# Autodesk Inventor assembly: NUEVO Ensamble de estructura H
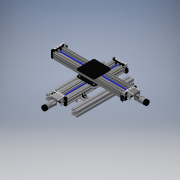
[picture p0: Inventor's stored thumbnail of the model, 180x180]
Saved by Autodesk Inventor 2018.3 (Build 223284000, 284)
## iProperties
Created: 2020-12-03
Part Number: NUEVO Ensamble de estructura H
Material: Genérico
Description: STEP AP203
Document SubType Name: Assembly
Designer: SERGIO ROMO
Sending System: SolidWorks 2019
Preprocessor: SwSTEP 2.0
Title: Ensamble del Arreglo.STEP
Revision Number: ANY
## Documents named in this file (23)
- C:\Users\SERGIO ROMO\Documents\GitHub\RemBot\CAD\Balanceo de masa\Inventor\NUEVO Ensamble de estructura H.iam
- C:\Users\SERGIO ROMO\Documents\GitHub\RemBot\CAD\Balanceo de masa\Inventor\C-Beam Actuator Lineal 500mm (Sin motor, sin carrito).ipt
- C:\Users\SERGIO ROMO\Documents\GitHub\RemBot\CAD\Balanceo de masa\Inventor\XLarge C-Beam Gantry Kit.iam
- C:\Users\SERGIO ROMO\Documents\GitHub\RemBot\CAD\Balanceo de masa\Inventor\Perfil de Aluminio.ipt
- C:\Users\SERGIO ROMO\Documents\GitHub\RemBot\CAD\Balanceo de masa\Inventor\Clavo.ipt
- C:\Users\SERGIO ROMO\Documents\GitHub\RemBot\CAD\Balanceo de masa\Inventor\Gearmotor_37D_19a1.ipt
- C:\Users\SERGIO ROMO\Documents\GitHub\RemBot\CAD\Balanceo de masa\Inventor\Impresion3D.ipt
- C:\Users\SERGIO ROMO\Documents\GitHub\RemBot\CAD\Balanceo de masa\Inventor\C-Beam Gantry Plate XLarge.step.ipt
- C:\Users\SERGIO ROMO\Documents\GitHub\RemBot\CAD\Balanceo de masa\Inventor\Bracket Inventor.ipt
- C:\Users\SERGIO ROMO\Documents\GitHub\RemBot\CAD\Balanceo de masa\Inventor\KW8-2.ipt
- C:\Users\SERGIO ROMO\Documents\GitHub\RemBot\CAD\Balanceo de masa\Inventor\Impresion3D sin Bracket.ipt
- C:\Users\SERGIO ROMO\Documents\GitHub\RemBot\CAD\Balanceo de masa\Inventor\Clavo de Arriba.ipt
- C:\Users\SERGIO ROMO\Documents\GitHub\RemBot\CAD\Balanceo de masa\Inventor\Tornillo final de carrera.ipt
- C:\Users\SERGIO ROMO\Documents\GitHub\RemBot\CAD\Balanceo de masa\Inventor\Perfil de Aluminio corta.ipt
- C:\Users\SERGIO ROMO\Documents\GitHub\RemBot\CAD\Balanceo de masa\Inventor\Triangulo.ipt
- C:\Users\SERGIO ROMO\Documents\GitHub\RemBot\CAD\Balanceo de masa\Inventor\TornilloM6.ipt
- C:\Users\SERGIO ROMO\Documents\GitHub\RemBot\CAD\Balanceo de masa\Inventor\Tuerca para tornilloM6.ipt
- C:\Users\SERGIO ROMO\Documents\GitHub\RemBot\CAD\Balanceo de masa\Inventor\Sujetador.ipt
- C:\Users\SERGIO ROMO\Documents\GitHub\RemBot\CAD\Balanceo de masa\Inventor\TornilloM8.ipt
- C:\Users\SERGIO ROMO\Documents\GitHub\RemBot\CAD\Balanceo de masa\Inventor\Tuerca para tornilloM8.ipt
- C:\Users\SERGIO ROMO\Documents\GitHub\RemBot\CAD\Balanceo de masa\Inventor\Tornillo para Bracket.ipt
- C:\Users\SERGIO ROMO\Documents\GitHub\RemBot\CAD\Balanceo de masa\Inventor\Tornillo para Motor Pololu.ipt
- C:\Users\SERGIO ROMO\Documents\GitHub\RemBot\CAD\Balanceo de masa\Inventor\Husillo 400 mm.ipt
## Components (100 placed, 27 different names)
1. XLarge C-Beam Gantry Kit_2 [sub-assembly] — Rígido:1
2. Perfil de Aluminio_4 — Coincidencia:37, Coincidencia:44, Coincidencia:60, Coincidencia:61, Coincidencia:75, Coincidencia:77
3. Perfil de Aluminio_5 — Coincidencia:36, Coincidencia:40, Coincidencia:64, Coincidencia:66, Coincidencia:79, Coincidencia:81
4. Clavo_8
5. Clavo_9
6. Gearmotor_37D_19a1_10 — Coincidencia:146
7. Gearmotor_37D_19a1_22
8. Impresion3D_28 — Coincidencia:1, Coincidencia:4, Coincidencia:15, Coincidencia:16, Coincidencia:28, Coincidencia:29, Coincidencia:30, Coincidencia:31, Coincidencia:83, Coincidencia:84, Coincidencia:147
9. C-Beam Actuator Lineal 500mm (Sin motor, sin carrito):2 — Rígido:1, Coincidencia:2, Coincidencia:9, Coincidencia:10
10. C-Beam Gantry Plate XLarge.step:1
11. Bracket Inventor:1 — Coincidencia:1, Coincidencia:83, Coincidencia:84, Coincidencia:106, Coincidencia:107, Coincidencia:108, Coincidencia:109, Coincidencia:110, Coincidencia:111, Coincidencia:112, Coincidencia:113, Coincidencia:134, Coincidencia:135, Coincidencia:136, Coincidencia:137, Coincidencia:138, Coincidencia:139, Coincidencia:140, Coincidencia:141, Coincidencia:142, Coincidencia:143, Coincidencia:144, Coincidencia:145
12. Bracket Inventor:2 — Coincidencia:3, Coincidencia:11, Coincidencia:12, Coincidencia:85, Coincidencia:114, Coincidencia:115, Coincidencia:116, Coincidencia:117, Coincidencia:118, Coincidencia:119, Coincidencia:120, Coincidencia:121, Coincidencia:122, Coincidencia:123, Coincidencia:124, Coincidencia:125, Coincidencia:126, Coincidencia:127, Coincidencia:128, Coincidencia:129, Coincidencia:130, Coincidencia:131, Coincidencia:132, Coincidencia:133
13. Impresion3D:2 — Coincidencia:2, Coincidencia:3, Coincidencia:5, Coincidencia:11, Coincidencia:12, Coincidencia:13, Coincidencia:14, Coincidencia:24, Coincidencia:25, Coincidencia:26, Coincidencia:27, Coincidencia:85, Coincidencia:90, Coincidencia:91, Coincidencia:92, Coincidencia:93
14. KW8-2:1 — Coincidencia:4
15. KW8-2:2 — Coincidencia:5
16. KW8-2:3 — Coincidencia:150
17. KW8-2:4
18. Impresion3D sin Bracket:1 — Coincidencia:17, Coincidencia:18, Coincidencia:19, Coincidencia:86, Coincidencia:87, Coincidencia:88, Coincidencia:89, Coincidencia:148, Coincidencia:149, Coincidencia:150, Coincidencia:151
19. Impresion3D sin Bracket:2 — Coincidencia:9, Coincidencia:10, Coincidencia:20, Coincidencia:21, Coincidencia:22, Coincidencia:23, Coincidencia:94, Coincidencia:95, Coincidencia:96, Coincidencia:97
20. Clavo:3 — Coincidencia:13
21. Clavo:4 — Coincidencia:14
22. Clavo de Arriba:1 — Coincidencia:15
23. Clavo de Arriba:2 — Coincidencia:16
24. Clavo de Arriba:3 — Coincidencia:17
25. Clavo de Arriba:4 — Coincidencia:18, Coincidencia:19
26. Clavo de Arriba:5 — Coincidencia:21, Coincidencia:23
27. Clavo de Arriba:6 — Coincidencia:20, Coincidencia:22
28. Clavo de Arriba:7 — Coincidencia:24, Coincidencia:25
29. Clavo de Arriba:8 — Coincidencia:26, Coincidencia:27
30. Tornillo final de carrera:1 — Coincidencia:28, Coincidencia:30
31. Tornillo final de carrera:2 — Coincidencia:29, Coincidencia:31
32. Perfil de Aluminio corta:1 — Coincidencia:37, Coincidencia:46, Coincidencia:55, Coincidencia:62, Coincidencia:63, Coincidencia:71, Coincidencia:72
33. Perfil de Aluminio corta:2 — Coincidencia:36, Coincidencia:38, Coincidencia:43, Coincidencia:51, Coincidencia:56, Coincidencia:59, Coincidencia:65, Coincidencia:67, Coincidencia:68
34. Triangulo:1 — Coincidencia:40, Coincidencia:47, Coincidencia:49, Coincidencia:102, Coincidencia:104
35. Triangulo:2 — Coincidencia:43, Coincidencia:53, Coincidencia:98, Coincidencia:100
36. Triangulo:3 — Coincidencia:38, Coincidencia:50, Coincidencia:103, Coincidencia:105
37. Triangulo:4 — Coincidencia:44, Coincidencia:54, Coincidencia:99, Coincidencia:101
38. TornilloM6:1 — Coincidencia:46, Coincidencia:47, Coincidencia:48
39. Tuerca para tornilloM6:1 — Coincidencia:48, Coincidencia:49
40. TornilloM6:2 — Coincidencia:50, Coincidencia:51, Coincidencia:52
41. Tuerca para tornilloM6:2 — Coincidencia:52
42. TornilloM6:3 — Coincidencia:53, Coincidencia:56, Coincidencia:57
43. TornilloM6:4 — Coincidencia:54, Coincidencia:55, Coincidencia:58
44. Tuerca para tornilloM6:3 — Coincidencia:57
45. Tuerca para tornilloM6:4 — Coincidencia:58
46. Sujetador:1 — Coincidencia:59, Coincidencia:60
47. Sujetador:2 — Coincidencia:61, Coincidencia:62
48. Sujetador:3 — Coincidencia:65, Coincidencia:66
49. Sujetador:4 — Coincidencia:63, Coincidencia:64
50. TornilloM8:1 — Coincidencia:68, Coincidencia:70
51. TornilloM8:2 — Coincidencia:67, Coincidencia:69
52. Tuerca para tornilloM8:1 — Coincidencia:69
53. Tuerca para tornilloM8:2 — Coincidencia:70
54. TornilloM8:3 — Coincidencia:71, Coincidencia:74
55. TornilloM8:4 — Coincidencia:72, Coincidencia:73
56. Tuerca para tornilloM8:3 — Coincidencia:73
57. Tuerca para tornilloM8:4 — Coincidencia:74
58. TornilloM8:5 — Coincidencia:75, Coincidencia:76
59. TornilloM8:6 — Coincidencia:77, Coincidencia:78
60. Tuerca para tornilloM8:5 — Coincidencia:76
61. Tuerca para tornilloM8:6 — Coincidencia:78
62. TornilloM8:7 — Coincidencia:81, Coincidencia:82
63. TornilloM8:8 — Coincidencia:79, Coincidencia:80
64. Tuerca para tornilloM8:7 — Coincidencia:80
65. Tuerca para tornilloM8:8 — Coincidencia:82
66. Tornillo final de carrera:3 — Coincidencia:86, Coincidencia:88, Coincidencia:151
67. Tornillo final de carrera:4 — Coincidencia:87, Coincidencia:89
68. Tornillo final de carrera:5 — Coincidencia:90, Coincidencia:92
69. Tornillo final de carrera:6 — Coincidencia:91, Coincidencia:93
70. Tornillo final de carrera:7 — Coincidencia:94, Coincidencia:96
71. Tornillo final de carrera:8 — Coincidencia:95, Coincidencia:97
72. TornilloM6:5 — Coincidencia:98
73. TornilloM6:6 — Coincidencia:99
74. Tuerca para tornilloM6:5 — Coincidencia:100
75. Tuerca para tornilloM6:6 — Coincidencia:101
76. TornilloM6:7 — Coincidencia:102
77. TornilloM6:8 — Coincidencia:103
78. Tuerca para tornilloM6:7 — Coincidencia:105
79. Tuerca para tornilloM6:8 — Coincidencia:104
80. Tornillo para Bracket:1 — Coincidencia:107, Coincidencia:111
81. Tornillo para Bracket:2 — Coincidencia:108, Coincidencia:112
82. Tornillo para Bracket:3 — Coincidencia:109, Coincidencia:110
83. Tornillo para Bracket:4 — Coincidencia:106, Coincidencia:113
84. Tornillo para Bracket:5 — Coincidencia:116, Coincidencia:121
85. Tornillo para Bracket:6 — Coincidencia:115, Coincidencia:118
86. Tornillo para Bracket:7 — Coincidencia:117, Coincidencia:120
87. Tornillo para Bracket:8 — Coincidencia:114, Coincidencia:119
88. Tornillo para Motor Pololu:1 — Coincidencia:127, Coincidencia:130
89. Tornillo para Motor Pololu:2 — Coincidencia:126, Coincidencia:128
90. Tornillo para Motor Pololu:3 — Coincidencia:124, Coincidencia:132
91. Tornillo para Motor Pololu:4 — Coincidencia:123, Coincidencia:131
92. Tornillo para Motor Pololu:5 — Coincidencia:125, Coincidencia:129
93. Tornillo para Motor Pololu:6 — Coincidencia:122, Coincidencia:133
94. Tornillo para Motor Pololu:7 — Coincidencia:138, Coincidencia:144
95. Tornillo para Motor Pololu:8 — Coincidencia:137, Coincidencia:143
96. Tornillo para Motor Pololu:9 — Coincidencia:136, Coincidencia:145
97. Tornillo para Motor Pololu:10 — Coincidencia:134, Coincidencia:141
98. Tornillo para Motor Pololu:11 — Coincidencia:135, Coincidencia:140
99. Tornillo para Motor Pololu:12 — Coincidencia:139, Coincidencia:142
100. Husillo 400 mm:1 — Coincidencia:146, Coincidencia:147, Coincidencia:148, Coincidencia:149
## Relationships (141: Mate 140, WeldJoint 1)
- Rígido:1 [WeldJoint]: XLarge C-Beam Gantry Kit_2 ↔ C-Beam Actuator Lineal 500mm (Sin motor, sin carrito):2
- Coincidencia:1 [Mate]: Impresion3D_28 ↔ Bracket Inventor:1
- Coincidencia:2 [Mate]: C-Beam Actuator Lineal 500mm (Sin motor, sin carrito):2 ↔ Impresion3D:2
- Coincidencia:3 [Mate]: Bracket Inventor:2 ↔ Impresion3D:2
- Coincidencia:4 [Mate]: Impresion3D_28 ↔ KW8-2:1
- Coincidencia:5 [Mate]: Impresion3D:2 ↔ KW8-2:2
- Coincidencia:9 [Mate]: C-Beam Actuator Lineal 500mm (Sin motor, sin carrito):2 ↔ Impresion3D sin Bracket:2
- Coincidencia:10 [Mate]: C-Beam Actuator Lineal 500mm (Sin motor, sin carrito):2 ↔ Impresion3D sin Bracket:2
- Coincidencia:11 [Mate]: Bracket Inventor:2 ↔ Impresion3D:2
- Coincidencia:12 [Mate]: Bracket Inventor:2 ↔ Impresion3D:2
- Coincidencia:13 [Mate]: Impresion3D:2 ↔ Clavo:3
- Coincidencia:14 [Mate]: Impresion3D:2 ↔ Clavo:4
- Coincidencia:15 [Mate]: Impresion3D_28 ↔ Clavo de Arriba:1
- Coincidencia:16 [Mate]: Impresion3D_28 ↔ Clavo de Arriba:2
- Coincidencia:17 [Mate]: Impresion3D sin Bracket:1 ↔ Clavo de Arriba:3
- Coincidencia:18 [Mate]: Impresion3D sin Bracket:1 ↔ Clavo de Arriba:4
- Coincidencia:19 [Mate]: Impresion3D sin Bracket:1 ↔ Clavo de Arriba:4
- Coincidencia:20 [Mate]: Impresion3D sin Bracket:2 ↔ Clavo de Arriba:6
- Coincidencia:21 [Mate]: Impresion3D sin Bracket:2 ↔ Clavo de Arriba:5
- Coincidencia:22 [Mate]: Impresion3D sin Bracket:2 ↔ Clavo de Arriba:6
- Coincidencia:23 [Mate]: Impresion3D sin Bracket:2 ↔ Clavo de Arriba:5
- Coincidencia:24 [Mate]: Impresion3D:2 ↔ Clavo de Arriba:7
- Coincidencia:25 [Mate]: Impresion3D:2 ↔ Clavo de Arriba:7
- Coincidencia:26 [Mate]: Impresion3D:2 ↔ Clavo de Arriba:8
- Coincidencia:27 [Mate]: Impresion3D:2 ↔ Clavo de Arriba:8
- Coincidencia:28 [Mate]: Impresion3D_28 ↔ Tornillo final de carrera:1
- Coincidencia:29 [Mate]: Impresion3D_28 ↔ Tornillo final de carrera:2
- Coincidencia:30 [Mate]: Impresion3D_28 ↔ Tornillo final de carrera:1
- Coincidencia:31 [Mate]: Impresion3D_28 ↔ Tornillo final de carrera:2
- Coincidencia:36 [Mate]: Perfil de Aluminio_5 ↔ Perfil de Aluminio corta:2
- Coincidencia:37 [Mate]: Perfil de Aluminio_4 ↔ Perfil de Aluminio corta:1
- Coincidencia:38 [Mate]: Perfil de Aluminio corta:2 ↔ Triangulo:3
- Coincidencia:40 [Mate]: Perfil de Aluminio_5 ↔ Triangulo:1
- Coincidencia:43 [Mate]: Perfil de Aluminio corta:2 ↔ Triangulo:2
- Coincidencia:44 [Mate]: Perfil de Aluminio_4 ↔ Triangulo:4
- Coincidencia:46 [Mate]: Perfil de Aluminio corta:1 ↔ TornilloM6:1
- Coincidencia:47 [Mate]: Triangulo:1 ↔ TornilloM6:1
- Coincidencia:48 [Mate]: TornilloM6:1 ↔ Tuerca para tornilloM6:1
- Coincidencia:49 [Mate]: Triangulo:1 ↔ Tuerca para tornilloM6:1
- Coincidencia:50 [Mate]: Triangulo:3 ↔ TornilloM6:2
- Coincidencia:51 [Mate]: Perfil de Aluminio corta:2 ↔ TornilloM6:2
- Coincidencia:52 [Mate]: TornilloM6:2 ↔ Tuerca para tornilloM6:2
- Coincidencia:53 [Mate]: Triangulo:2 ↔ TornilloM6:3
- Coincidencia:54 [Mate]: Triangulo:4 ↔ TornilloM6:4
- Coincidencia:55 [Mate]: Perfil de Aluminio corta:1 ↔ TornilloM6:4
- Coincidencia:56 [Mate]: Perfil de Aluminio corta:2 ↔ TornilloM6:3
- Coincidencia:57 [Mate]: TornilloM6:3 ↔ Tuerca para tornilloM6:3
- Coincidencia:58 [Mate]: TornilloM6:4 ↔ Tuerca para tornilloM6:4
- Coincidencia:59 [Mate]: Perfil de Aluminio corta:2 ↔ Sujetador:1
- Coincidencia:60 [Mate]: Perfil de Aluminio_4 ↔ Sujetador:1
- Coincidencia:61 [Mate]: Perfil de Aluminio_4 ↔ Sujetador:2
- Coincidencia:62 [Mate]: Perfil de Aluminio corta:1 ↔ Sujetador:2
- Coincidencia:63 [Mate]: Perfil de Aluminio corta:1 ↔ Sujetador:4
- Coincidencia:64 [Mate]: Perfil de Aluminio_5 ↔ Sujetador:4
- Coincidencia:65 [Mate]: Perfil de Aluminio corta:2 ↔ Sujetador:3
- Coincidencia:66 [Mate]: Perfil de Aluminio_5 ↔ Sujetador:3
- Coincidencia:67 [Mate]: Perfil de Aluminio corta:2 ↔ TornilloM8:2
- Coincidencia:68 [Mate]: Perfil de Aluminio corta:2 ↔ TornilloM8:1
- Coincidencia:69 [Mate]: TornilloM8:2 ↔ Tuerca para tornilloM8:1
- Coincidencia:70 [Mate]: TornilloM8:1 ↔ Tuerca para tornilloM8:2
- Coincidencia:71 [Mate]: Perfil de Aluminio corta:1 ↔ TornilloM8:3
- Coincidencia:72 [Mate]: Perfil de Aluminio corta:1 ↔ TornilloM8:4
- Coincidencia:73 [Mate]: TornilloM8:4 ↔ Tuerca para tornilloM8:3
- Coincidencia:74 [Mate]: TornilloM8:3 ↔ Tuerca para tornilloM8:4
- Coincidencia:75 [Mate]: Perfil de Aluminio_4 ↔ TornilloM8:5
- Coincidencia:76 [Mate]: TornilloM8:5 ↔ Tuerca para tornilloM8:5
- Coincidencia:77 [Mate]: Perfil de Aluminio_4 ↔ TornilloM8:6
- Coincidencia:78 [Mate]: TornilloM8:6 ↔ Tuerca para tornilloM8:6
- Coincidencia:79 [Mate]: Perfil de Aluminio_5 ↔ TornilloM8:8
- Coincidencia:80 [Mate]: TornilloM8:8 ↔ Tuerca para tornilloM8:7
- Coincidencia:81 [Mate]: Perfil de Aluminio_5 ↔ TornilloM8:7
- Coincidencia:82 [Mate]: TornilloM8:7 ↔ Tuerca para tornilloM8:8
- Coincidencia:83 [Mate]: Impresion3D_28 ↔ Bracket Inventor:1
- Coincidencia:84 [Mate]: Impresion3D_28 ↔ Bracket Inventor:1
- Coincidencia:85 [Mate]: Bracket Inventor:2 ↔ Impresion3D:2
- Coincidencia:86 [Mate]: Impresion3D sin Bracket:1 ↔ Tornillo final de carrera:3
- Coincidencia:87 [Mate]: Impresion3D sin Bracket:1 ↔ Tornillo final de carrera:4
- Coincidencia:88 [Mate]: Impresion3D sin Bracket:1 ↔ Tornillo final de carrera:3
- Coincidencia:89 [Mate]: Impresion3D sin Bracket:1 ↔ Tornillo final de carrera:4
- Coincidencia:90 [Mate]: Impresion3D:2 ↔ Tornillo final de carrera:5
- Coincidencia:91 [Mate]: Impresion3D:2 ↔ Tornillo final de carrera:6
- Coincidencia:92 [Mate]: Impresion3D:2 ↔ Tornillo final de carrera:5
- Coincidencia:93 [Mate]: Impresion3D:2 ↔ Tornillo final de carrera:6
- Coincidencia:94 [Mate]: Impresion3D sin Bracket:2 ↔ Tornillo final de carrera:7
- Coincidencia:95 [Mate]: Impresion3D sin Bracket:2 ↔ Tornillo final de carrera:8
- Coincidencia:96 [Mate]: Impresion3D sin Bracket:2 ↔ Tornillo final de carrera:7
- Coincidencia:97 [Mate]: Impresion3D sin Bracket:2 ↔ Tornillo final de carrera:8
- Coincidencia:98 [Mate]: Triangulo:2 ↔ TornilloM6:5
- Coincidencia:99 [Mate]: Triangulo:4 ↔ TornilloM6:6
- Coincidencia:100 [Mate]: Triangulo:2 ↔ Tuerca para tornilloM6:5
- Coincidencia:101 [Mate]: Triangulo:4 ↔ Tuerca para tornilloM6:6
- Coincidencia:102 [Mate]: Triangulo:1 ↔ TornilloM6:7
- Coincidencia:103 [Mate]: Triangulo:3 ↔ TornilloM6:8
- Coincidencia:104 [Mate]: Triangulo:1 ↔ Tuerca para tornilloM6:8
- Coincidencia:105 [Mate]: Triangulo:3 ↔ Tuerca para tornilloM6:7
- Coincidencia:106 [Mate]: Bracket Inventor:1 ↔ Tornillo para Bracket:4
- Coincidencia:107 [Mate]: Bracket Inventor:1 ↔ Tornillo para Bracket:1
- Coincidencia:108 [Mate]: Bracket Inventor:1 ↔ Tornillo para Bracket:2
- Coincidencia:109 [Mate]: Bracket Inventor:1 ↔ Tornillo para Bracket:3
- Coincidencia:110 [Mate]: Bracket Inventor:1 ↔ Tornillo para Bracket:3
- Coincidencia:111 [Mate]: Bracket Inventor:1 ↔ Tornillo para Bracket:1
- Coincidencia:112 [Mate]: Bracket Inventor:1 ↔ Tornillo para Bracket:2
- Coincidencia:113 [Mate]: Bracket Inventor:1 ↔ Tornillo para Bracket:4
- Coincidencia:114 [Mate]: Bracket Inventor:2 ↔ Tornillo para Bracket:8
- Coincidencia:115 [Mate]: Bracket Inventor:2 ↔ Tornillo para Bracket:6
- Coincidencia:116 [Mate]: Bracket Inventor:2 ↔ Tornillo para Bracket:5
- Coincidencia:117 [Mate]: Bracket Inventor:2 ↔ Tornillo para Bracket:7
- Coincidencia:118 [Mate]: Bracket Inventor:2 ↔ Tornillo para Bracket:6
- Coincidencia:119 [Mate]: Bracket Inventor:2 ↔ Tornillo para Bracket:8
- Coincidencia:120 [Mate]: Bracket Inventor:2 ↔ Tornillo para Bracket:7
- Coincidencia:121 [Mate]: Bracket Inventor:2 ↔ Tornillo para Bracket:5
- Coincidencia:122 [Mate]: Bracket Inventor:2 ↔ Tornillo para Motor Pololu:6
- Coincidencia:123 [Mate]: Bracket Inventor:2 ↔ Tornillo para Motor Pololu:4
- Coincidencia:124 [Mate]: Bracket Inventor:2 ↔ Tornillo para Motor Pololu:3
- Coincidencia:125 [Mate]: Bracket Inventor:2 ↔ Tornillo para Motor Pololu:5
- Coincidencia:126 [Mate]: Bracket Inventor:2 ↔ Tornillo para Motor Pololu:2
- Coincidencia:127 [Mate]: Bracket Inventor:2 ↔ Tornillo para Motor Pololu:1
- Coincidencia:128 [Mate]: Bracket Inventor:2 ↔ Tornillo para Motor Pololu:2
- Coincidencia:129 [Mate]: Bracket Inventor:2 ↔ Tornillo para Motor Pololu:5
- Coincidencia:130 [Mate]: Bracket Inventor:2 ↔ Tornillo para Motor Pololu:1
- Coincidencia:131 [Mate]: Bracket Inventor:2 ↔ Tornillo para Motor Pololu:4
- Coincidencia:132 [Mate]: Bracket Inventor:2 ↔ Tornillo para Motor Pololu:3
- Coincidencia:133 [Mate]: Bracket Inventor:2 ↔ Tornillo para Motor Pololu:6
- Coincidencia:134 [Mate]: Bracket Inventor:1 ↔ Tornillo para Motor Pololu:10
- Coincidencia:135 [Mate]: Bracket Inventor:1 ↔ Tornillo para Motor Pololu:11
- Coincidencia:136 [Mate]: Bracket Inventor:1 ↔ Tornillo para Motor Pololu:9
- Coincidencia:137 [Mate]: Bracket Inventor:1 ↔ Tornillo para Motor Pololu:8
- Coincidencia:138 [Mate]: Bracket Inventor:1 ↔ Tornillo para Motor Pololu:7
- Coincidencia:139 [Mate]: Bracket Inventor:1 ↔ Tornillo para Motor Pololu:12
- Coincidencia:140 [Mate]: Bracket Inventor:1 ↔ Tornillo para Motor Pololu:11
- Coincidencia:141 [Mate]: Bracket Inventor:1 ↔ Tornillo para Motor Pololu:10
- Coincidencia:142 [Mate]: Bracket Inventor:1 ↔ Tornillo para Motor Pololu:12
- Coincidencia:143 [Mate]: Bracket Inventor:1 ↔ Tornillo para Motor Pololu:8
- Coincidencia:144 [Mate]: Bracket Inventor:1 ↔ Tornillo para Motor Pololu:7
- Coincidencia:145 [Mate]: Bracket Inventor:1 ↔ Tornillo para Motor Pololu:9
- Coincidencia:146 [Mate]: Gearmotor_37D_19a1_10 ↔ Husillo 400 mm:1
- Coincidencia:147 [Mate]: Impresion3D_28 ↔ Husillo 400 mm:1
- Coincidencia:148 [Mate]: Impresion3D sin Bracket:1 ↔ Husillo 400 mm:1
- Coincidencia:149 [Mate]: Impresion3D sin Bracket:1 ↔ Husillo 400 mm:1
- Coincidencia:150 [Mate]: KW8-2:3 ↔ Impresion3D sin Bracket:1
- Coincidencia:151 [Mate]: Impresion3D sin Bracket:1 ↔ Tornillo final de carrera:3
